# Autodesk Inventor assembly: Assem4
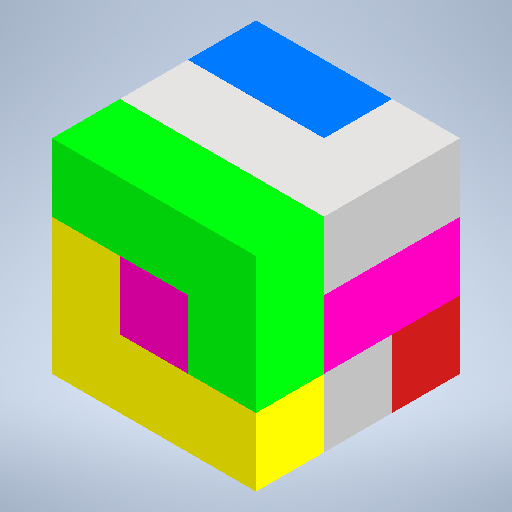
[picture p0: Inventor's stored thumbnail of the model, 512x512]
Saved by Autodesk Inventor 2025 (Build 290162000, 162)
## iProperties
Created: 2024-10-06
Part Number: Assem4
Description: STEP AP203
Document SubType Name: Assembly
Designer: dell
Title: Assem4.STEP
Revision Number: ANY
## Documents named in this file (5)
- C:\Users\dell\Desktop\2022,mc58\Semester5\Design of Machine Element\LAB\lab3\Assem4\Assem4.iam
- C:\Users\dell\Desktop\2022,mc58\Semester5\Design of Machine Element\LAB\lab3\task2Part1\task2Part1.ipt
- C:\Users\dell\Desktop\2022,mc58\Semester5\Design of Machine Element\LAB\lab3\task2Part2\task2Part2.ipt
- C:\Users\dell\Desktop\2022,mc58\Semester5\Design of Machine Element\LAB\lab3\task2Part3\task2Part3.ipt
- C:\Users\dell\Desktop\2022,mc58\Semester5\Design of Machine Element\LAB\lab3\task2part4\task2part4.ipt
## Components (7 placed, 4 different names)
1. task2Part1:1 — Rigid:1
2. task2Part2:1 — Rigid:4, Rigid:6
3. task2Part3:1 — Rigid:4
4. task2part4:1 — Rigid:2, Rigid:3, Rigid:5, Rigid:6
5. task2Part1:2 — Rigid:1, Rigid:5
6. task2Part1:3 — Rigid:2
7. task2Part1:4 — Rigid:3
## Relationships (6: WeldJoint 6)
- Rigid:1 [WeldJoint]: task2Part1:1 ↔ task2Part1:2
- Rigid:2 [WeldJoint]: task2part4:1 ↔ task2Part1:3
- Rigid:3 [WeldJoint]: task2part4:1 ↔ task2Part1:4
- Rigid:4 [WeldJoint]: task2Part2:1 ↔ task2Part3:1
- Rigid:5 [WeldJoint]: task2part4:1 ↔ task2Part1:2
- Rigid:6 [WeldJoint]: task2Part2:1 ↔ task2part4:1
